# Autodesk Inventor assembly: мультипликатор
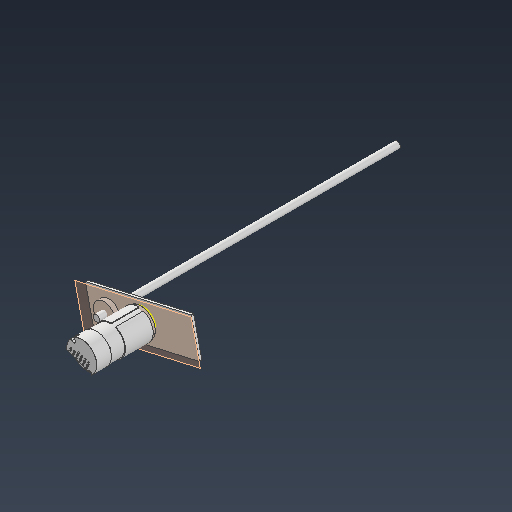
[picture p0: Inventor's stored thumbnail of the model, 512x512]
Saved by Autodesk Inventor 2025 (Build 290162000, 162)
## iProperties
Created: 2025-09-21
Part Number: мультипликатор
Document SubType Name: Assembly
Designer: GameHD
Author: GameHD
## Documents named in this file (5)
- C:\Users\GameHD\Desktop\Phantom 16950\мультипликатор.iam
- C:\Users\GameHD\Desktop\Phantom 16950\мультипликатор\Мастер проектирования\Цилиндрическое зубчатое зацепление3.iam
- C:\Users\GameHD\Desktop\Phantom 16950\пластина для редуктора.ipt
- C:\Users\GameHD\Desktop\Phantom 16950\5000-0002-0117\5000-0002-0117.iam
- C:\Users\GameHD\Desktop\Phantom 16950\вал кб.ipt
## Components (5 placed, 4 different names)
1. Цилиндрическое зубчатое зацепление:2 [sub-assembly] — Заподлицо:1, Совмещение:3, Заподлицо:2
2. пластина для редуктора:1 — Совмещение:1, Совмещение:2, Совмещение:3, Совмещение:4
3. 5000-0002-0117:2 [sub-assembly] — Заподлицо:1, Совмещение:1, Совмещение:2
4. Цилиндрическое зубчатое зацепление:3 [sub-assembly] — Совмещение:4, Заподлицо:2, Совмещение:5
5. вал кб:1 — Совмещение:5
## Relationships (7: Mate 5, Flush 2)
- Заподлицо:1 [Flush]: Цилиндрическое зубчатое зацепление:2 ↔ 5000-0002-0117:2
- Совмещение:1 [Mate]: пластина для редуктора:1 ↔ 5000-0002-0117:2
- Совмещение:2 [Mate]: пластина для редуктора:1 ↔ 5000-0002-0117:2
- Совмещение:3 [Mate]: Цилиндрическое зубчатое зацепление:2 ↔ пластина для редуктора:1
- Совмещение:4 [Mate]: пластина для редуктора:1 ↔ Цилиндрическое зубчатое зацепление:3
- Заподлицо:2 [Flush]: Цилиндрическое зубчатое зацепление:2 ↔ Цилиндрическое зубчатое зацепление:3
- Совмещение:5 [Mate]: Цилиндрическое зубчатое зацепление:3 ↔ вал кб:1
